# Autodesk Inventor assembly: EV-ADL5534
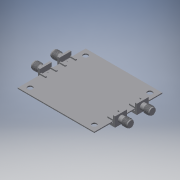
[picture p0: Inventor's stored thumbnail of the model, 180x180]
Saved by Autodesk Inventor 2018 (Build 220112000, 112)
## iProperties
Created: 2018-04-06
Part Number: EV-ADL5534
Document SubType Name: Assembly
Designer: bbramman
Author: bbramman
## Documents named in this file (3)
- C:\Users\bbramman\OneDrive\Documents\Trapped Ion Research (Grad)\Electronics\pll-evalboard-synthesizer\Box CAD\EV-ADL5534.iam
- C:\Users\bbramman\OneDrive\Documents\Trapped Ion Research (Grad)\Electronics\pll-evalboard-synthesizer\Box CAD\62x55mm-PCB.ipt
- C:\Users\bbramman\OneDrive\Documents\Trapped Ion Research (Grad)\Electronics\pll-evalboard-synthesizer\Box CAD\SMA-END.ipt
## Components (5 placed, 2 different names)
1. 62x55mm-PCB:1 — Mate:1, Mate:2, Mate:3, Mate:4, Mate:5, Mate:6, Mate:7, Mate:8
2. SMA-END:1 — Mate:2, Mate:3
3. SMA-END:2 — Mate:1, Mate:4
4. SMA-END:3 — Mate:7, Mate:8
5. SMA-END:4 — Mate:5, Mate:6
## Relationships (8: Mate 8)
- Mate:1: 62x55mm-PCB:1 ↔ SMA-END:2
- Mate:2: 62x55mm-PCB:1 ↔ SMA-END:1
- Mate:3: 62x55mm-PCB:1 ↔ SMA-END:1
- Mate:4: 62x55mm-PCB:1 ↔ SMA-END:2
- Mate:5: 62x55mm-PCB:1 ↔ SMA-END:4
- Mate:6: 62x55mm-PCB:1 ↔ SMA-END:4
- Mate:7: 62x55mm-PCB:1 ↔ SMA-END:3
- Mate:8: 62x55mm-PCB:1 ↔ SMA-END:3
